# Autodesk Inventor assembly: Drone Assembly
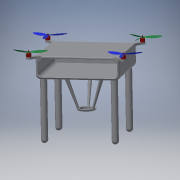
[picture p0: Inventor's stored thumbnail of the model, 180x180]
Saved by Autodesk Inventor 2019 (Build 230136000, 136)
## iProperties
Created: 2020-03-20
Part Number: Drone Assembly
Document SubType Name: Assembly
Designer: 18186
Author: 18186
## Documents named in this file (7)
- D:\Food Delivery Drone\Drone Assembly.iam
- D:\Food Delivery Drone\Drone Body.ipt
- D:\Food Delivery Drone\motor mock.ipt
- D:\Food Delivery Drone\PropellerCW-3Blade.ipt
- D:\Food Delivery Drone\Drone Body Cupholder.ipt
- D:\Food Delivery Drone\Drone Body Leg.ipt
- D:\Food Delivery Drone\PropellerCCW-3Blade.ipt
## Components (14 placed, 6 different names)
1. Drone Body:1 — Mate:17, Mate:18, Mate:19, Mate:20, Mate:21, Mate:22, Mate:23, Mate:24, Mate:29, Tangent:1, Mate:30, Mate:31, Mate:32, Mate:43, Mate:44, Mate:45, Mate:46, Mate:47, Mate:48
2. motor mock:1 — Mate:21, Mate:22, Mate:27, Mate:28
3. motor mock:2 — Mate:17, Mate:18, Mate:25, Mate:26
4. motor mock:3 — Mate:19, Mate:20, Mate:41, Mate:42
5. motor mock:4 — Mate:23, Mate:24, Mate:39, Mate:40
6. PropellerCW-3Blade:1 — Mate:27, Mate:28
7. PropellerCW-3Blade:2 — Mate:25, Mate:26
8. Drone Body Cupholder:1 — Mate:29, Tangent:1, Mate:30
9. Drone Body Leg:3 — Mate:31, Mate:32
10. PropellerCCW-3Blade:1 — Mate:39, Mate:40
11. PropellerCCW-3Blade:2 — Mate:41, Mate:42
12. Drone Body Leg:4 — Mate:43, Mate:44
13. Drone Body Leg:5 — Mate:45, Mate:47
14. Drone Body Leg:6 — Mate:46, Mate:48
## Relationships (27: Mate 26, Tangent 1)
- Mate:17: Drone Body:1 ↔ motor mock:2
- Mate:18: Drone Body:1 ↔ motor mock:2
- Mate:19: Drone Body:1 ↔ motor mock:3
- Mate:20: Drone Body:1 ↔ motor mock:3
- Mate:21: Drone Body:1 ↔ motor mock:1
- Mate:22: Drone Body:1 ↔ motor mock:1
- Mate:23: Drone Body:1 ↔ motor mock:4
- Mate:24: Drone Body:1 ↔ motor mock:4
- Mate:25: motor mock:2 ↔ PropellerCW-3Blade:2
- Mate:26: motor mock:2 ↔ PropellerCW-3Blade:2
- Mate:27: motor mock:1 ↔ PropellerCW-3Blade:1
- Mate:28: motor mock:1 ↔ PropellerCW-3Blade:1
- Mate:29: Drone Body:1 ↔ Drone Body Cupholder:1
- Tangent:1: Drone Body:1 ↔ Drone Body Cupholder:1
- Mate:30: Drone Body:1 ↔ Drone Body Cupholder:1
- Mate:31: Drone Body:1 ↔ Drone Body Leg:3
- Mate:32: Drone Body:1 ↔ Drone Body Leg:3
- Mate:39: motor mock:4 ↔ PropellerCCW-3Blade:1
- Mate:40: motor mock:4 ↔ PropellerCCW-3Blade:1
- Mate:41: motor mock:3 ↔ PropellerCCW-3Blade:2
- Mate:42: motor mock:3 ↔ PropellerCCW-3Blade:2
- Mate:43: Drone Body:1 ↔ Drone Body Leg:4
- Mate:44: Drone Body:1 ↔ Drone Body Leg:4
- Mate:45: Drone Body:1 ↔ Drone Body Leg:5
- Mate:46: Drone Body:1 ↔ Drone Body Leg:6
- Mate:47: Drone Body:1 ↔ Drone Body Leg:5
- Mate:48: Drone Body:1 ↔ Drone Body Leg:6
